# Autodesk Inventor assembly: Kit Frame 28x38 Long JB
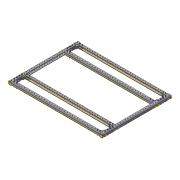
[picture p0: Inventor's stored thumbnail of the model, 180x180]
Saved by Autodesk Inventor 2013 (Build 170138000, 138)
## iProperties
Created: 2013-04-20
Part Number: Kit Frame 28x38 Long JB
Document SubType Name: Assembly
Designer: niemitalo_dan
Author: niemitalo_dan
## Documents named in this file (4)
- \\lmss\students\Robotics\CAD Files\COTS Parts\Kit Frame - AndyMark\Kit Frame 28x38 Long JB.iam
- \\lmss\students\Robotics\CAD Files\COTS Parts\Kit Frame - AndyMark\C Channel.ipt
- \\lmss\students\Robotics\CAD Files\COTS Parts\Kit Frame - AndyMark\Components\C Channel Short for Long Base.ipt
- \\lmss\students\Robotics\CAD Files\COTS Parts\Kit Frame - AndyMark\Components\CornerConnectAssyLeft.iam
## Components (14 placed, 3 different names)
1. C Channel:1 — Flush:1, Flush:2, Flush:3, Flush:5, Mate:1, Insert:1, Insert:7, Flush:7, Mate:4, Flush:8, Flush:9
2. C Channel:2 — Flush:5, Mate:1, Insert:3, Insert:5
3. C Channel:3 — Flush:7, Mate:4, Insert:9, Insert:13
4. C Channel:4 — Flush:8, Flush:9, Insert:11, Insert:15
5. C Channel Short for Long Base:1 — Flush:3, Flush:4, Flush:6, Mate:2, Insert:2, Mate:3, Insert:4, Insert:10, Insert:12
6. C Channel Short for Long Base:2 — Flush:6, Mate:2, Insert:6, Insert:8, Insert:14, Insert:16
7. CornerConnectAssyLeft:1 [sub-assembly] — Insert:1, Insert:2, Mate:3
8. CornerConnectAssyLeft:2 [sub-assembly] — Insert:3, Insert:4
9. CornerConnectAssyLeft:3 [sub-assembly] — Insert:5, Insert:6
10. CornerConnectAssyLeft:4 [sub-assembly] — Insert:7, Insert:8
11. CornerConnectAssyLeft:5 [sub-assembly] — Insert:9, Insert:10
12. CornerConnectAssyLeft:6 [sub-assembly] — Insert:11, Insert:12
13. CornerConnectAssyLeft:7 [sub-assembly] — Insert:13, Insert:14
14. CornerConnectAssyLeft:8 [sub-assembly] — Insert:15, Insert:16
## Relationships (29: Insert 16, Flush 9, Mate 4)
- Flush:1: C Channel:1
- Flush:2: C Channel:1
- Flush:3: C Channel:1 ↔ C Channel Short for Long Base:1
- Flush:4: C Channel Short for Long Base:1
- Flush:5: C Channel:1 ↔ C Channel:2
- Mate:1: C Channel:1 ↔ C Channel:2
- Flush:6: C Channel Short for Long Base:1 ↔ C Channel Short for Long Base:2
- Mate:2: C Channel Short for Long Base:1 ↔ C Channel Short for Long Base:2
- Insert:1: C Channel:1 ↔ CornerConnectAssyLeft:1
- Insert:2: C Channel Short for Long Base:1 ↔ CornerConnectAssyLeft:1
- Mate:3: C Channel Short for Long Base:1 ↔ CornerConnectAssyLeft:1
- Insert:3: C Channel:2 ↔ CornerConnectAssyLeft:2
- Insert:4: C Channel Short for Long Base:1 ↔ CornerConnectAssyLeft:2
- Insert:5: C Channel:2 ↔ CornerConnectAssyLeft:3
- Insert:6: C Channel Short for Long Base:2 ↔ CornerConnectAssyLeft:3
- Insert:7: C Channel:1 ↔ CornerConnectAssyLeft:4
- Insert:8: C Channel Short for Long Base:2 ↔ CornerConnectAssyLeft:4
- Flush:7: C Channel:1 ↔ C Channel:3
- Mate:4: C Channel:1 ↔ C Channel:3
- Flush:8: C Channel:1 ↔ C Channel:4
- Flush:9: C Channel:1 ↔ C Channel:4
- Insert:9: C Channel:3 ↔ CornerConnectAssyLeft:5
- Insert:10: C Channel Short for Long Base:1 ↔ CornerConnectAssyLeft:5
- Insert:11: C Channel:4 ↔ CornerConnectAssyLeft:6
- Insert:12: C Channel Short for Long Base:1 ↔ CornerConnectAssyLeft:6
- Insert:13: C Channel:3 ↔ CornerConnectAssyLeft:7
- Insert:14: C Channel Short for Long Base:2 ↔ CornerConnectAssyLeft:7
- Insert:15: C Channel:4 ↔ CornerConnectAssyLeft:8
- Insert:16: C Channel Short for Long Base:2 ↔ CornerConnectAssyLeft:8
